# Autodesk Inventor assembly: Shifting Cylinder Mechanism for Ball Shifter
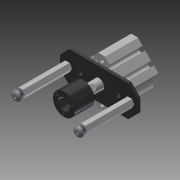
[picture p0: Inventor's stored thumbnail of the model, 180x180]
Saved by Autodesk Inventor 2013 (Build 170138000, 138)
## iProperties
Created: 2013-04-08
Part Number: Shifting Cylinder Mechanism for Ball Shifter
Document SubType Name: Assembly
Designer: Niemitalo_Dan
Author: Niemitalo_Dan
## Documents named in this file (8)
- \\lmss\STUDENTS\Robotics\CAD Files\COTS Parts\Gearboxes\Components\VexPro Ballshifter Components\Shifting Cylinder Mechanism for Ball Shifter.iam
- \\lmss\STUDENTS\Robotics\CAD Files\COTS Parts\Fasteners\Hex Standoff 8-32 x1500.ipt
- \\lmss\STUDENTS\Robotics\CAD Files\COTS Parts\Fasteners\8-32 BHCS x375.ipt
- \\lmss\STUDENTS\Robotics\CAD Files\COTS Parts\Gearboxes\Ball Shifter\BS cylinder mounting plate.ipt
- \\lmss\STUDENTS\Robotics\CAD Files\COTS Parts\Gearboxes\Components\VexPro Ballshifter Components\Ballshifter Cylinder.iam
- \\lmss\STUDENTS\Robotics\CAD Files\COTS Parts\Gearboxes\Components\VexPro Ballshifter Components\Jam Nut for Ballshifter Cylinder.ipt
- \\lmss\STUDENTS\Robotics\CAD Files\COTS Parts\Gearboxes\Ball Shifter\Ball Shifter shifter coupling side 1.ipt
- \\lmss\STUDENTS\Robotics\CAD Files\COTS Parts\Gearboxes\Ball Shifter\Ball Shifter shifter coupling side 2.ipt
## Components (11 placed, 7 different names)
1. Hex Standoff 8-32 x1500:1 — Insert:6, Angle:4
2. Hex Standoff 8-32 x1500:2 — Insert:5, Mate:3, Angle:2, Angle:5
3. 8-32 BHCS x375:1 — Insert:6
4. 8-32 BHCS x375:2 — Insert:5
5. BS cylinder mounting plate:1 — Mate:3, Angle:4, Angle:5
6. 8-32 BHCS x375:3
7. 8-32 BHCS x375:4
8. Ballshifter Cylinder:1 [sub-assembly] — Mate:2, Flush:1, Mate:4, Mate:5, Angle:3
9. Jam Nut for Ballshifter Cylinder:1 — Mate:2, Flush:1, Mate:7, Angle:2
10. Ball Shifter shifter coupling side 1:1 — Mate:5, Mate:6, Mate:7, Flush:2, Angle:3
11. Ball Shifter shifter coupling side 2:1 — Mate:4, Mate:6, Flush:2
## Relationships (20: Mate 7, Insert 6, Angle 5, Flush 2)
- [Insert]: Hex Standoff 8-32 x1500:1 ↔ BS cylinder mounting plate:1
- [Mate]: Hex Standoff 8-32 x1500:2 ↔ BS cylinder mounting plate:1
- [Insert]: BS cylinder mounting plate:1 ↔ 8-32 BHCS x375:3
- [Insert]: BS cylinder mounting plate:1 ↔ 8-32 BHCS x375:4
- [Insert]: BS cylinder mounting plate:1 ↔ Ballshifter Cylinder:1
- [Angle] (45 deg): BS cylinder mounting plate:1 ↔ Ballshifter Cylinder:1
- Mate:2: Ballshifter Cylinder:1 ↔ Jam Nut for Ballshifter Cylinder:1
- Insert:5 (3.175 mm): Hex Standoff 8-32 x1500:2 ↔ 8-32 BHCS x375:2
- Insert:6 (3.175 mm): Hex Standoff 8-32 x1500:1 ↔ 8-32 BHCS x375:1
- Mate:3: Hex Standoff 8-32 x1500:2 ↔ BS cylinder mounting plate:1
- Flush:1: Ballshifter Cylinder:1 ↔ Jam Nut for Ballshifter Cylinder:1
- Mate:4: Ballshifter Cylinder:1 ↔ Ball Shifter shifter coupling side 2:1
- Mate:5: Ballshifter Cylinder:1 ↔ Ball Shifter shifter coupling side 1:1
- Mate:6: Ball Shifter shifter coupling side 1:1 ↔ Ball Shifter shifter coupling side 2:1
- Mate:7: Jam Nut for Ballshifter Cylinder:1 ↔ Ball Shifter shifter coupling side 1:1
- Flush:2: Ball Shifter shifter coupling side 1:1 ↔ Ball Shifter shifter coupling side 2:1
- Angle:2 (0 deg): Hex Standoff 8-32 x1500:2 ↔ Jam Nut for Ballshifter Cylinder:1
- Angle:3 (0 deg): Ballshifter Cylinder:1 ↔ Ball Shifter shifter coupling side 1:1
- Angle:4 (0 deg): Hex Standoff 8-32 x1500:1 ↔ BS cylinder mounting plate:1
- Angle:5 (0 deg): Hex Standoff 8-32 x1500:2 ↔ BS cylinder mounting plate:1
